# Autodesk Inventor assembly: Assembly1
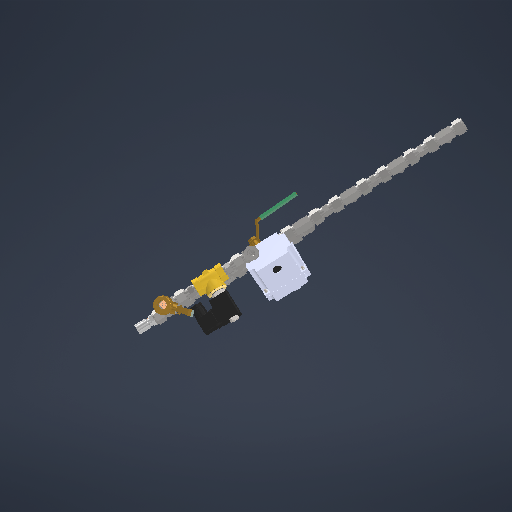
[picture p0: Inventor's stored thumbnail of the model, 512x512]
Saved by Autodesk Inventor 2026.2 (Build 302298000, 298)
## iProperties
Created: 2026-01-25
Part Number: Assembly1
Document SubType Name: Assembly
Designer: szwed
Author: szwed
## Documents named in this file (9)
- C:\Users\szwed\Desktop\R7\Assembly1.iam
- C:\Users\szwed\Documents\Inventor\Content Center Files\R2026\en-US\ISO 49 N8\ISO 49 Hexagon Nipple N8 3_8.ipt
- C:\Users\szwed\Documents\Inventor\Content Center Files\R2026\en-US\Parker A(16)\Parker A-Lok - Fractional Tube 1_2 (4).ipt
- C:\Users\szwed\Documents\Inventor\Content Center Files\R2026\en-US\Parker A(01)\Parker A-Lok - Metric to Inch Tube 12 x 1_2.ipt
- C:\Users\szwed\Documents\Inventor\Content Center Files\R2026\en-US\Parker A-Lok - 90deg Elbow - Fractional Tube\1_2(37).ipt
- C:\Users\szwed\Desktop\gs_solidworks-master\R7_GS_1110_SERVOVALVE\R7_GS_1110_SERVOVALVE\R7_GS_1110_SERVOVALVE\R7_GS_1110_SERVOVALVE.ipt
- C:\Users\szwed\Documents\Inventor\Content Center Files\R2026\en-US\Parker XV500P\Parker Female-Female Pipe Ends XV500P XV500P-8.ipt
- C:\Users\szwed\Documents\Inventor\Content Center Files\R2026\en-US\Parker MTT 2\Parker Male Taper Thread 1_4 x 3_8.ipt
- C:\Users\szwed\Downloads\MV04_DN8_3-8 Zoll\MV04_DN8_3-8 Zoll\MV04_DN8_3-8 Zoll.ipt
## Components (38 placed, 8 different names)
1. ISO 49 Hexagon Nipple N8 3/8:1 — Insert:7, Insert:8
2. Parker A-Lok - Fractional Tube 1/2:1 — Insert:2, Flush:1, Insert:3, Flush:2
3. ISO 49 Hexagon Nipple N8 3/8:5 — Insert:5, Insert:6
4. Parker A-Lok - Fractional Tube 1/2:2 — Insert:10, Flush:4, Insert:12, Insert:22, Flush:5, Flush:6
5. ISO 49 Hexagon Nipple N8 3/8:6 — Insert:15, Insert:17
6. Parker A-Lok - Fractional Tube 1/2:3 — Insert:4, Insert:5, Flush:2, Flush:3
7. ISO 49 Hexagon Nipple N8 3/8:7 — Insert:1, Insert:2
8. Parker A-Lok - Fractional Tube 1/2:4 — Insert:1, Flush:1
9. Parker A-Lok - Metric to Inch Tube 12 x 1/2:1 — Insert:13, Insert:15
10. ISO 49 Hexagon Nipple N8 3/8:8 — Insert:31, Insert:32
11. ISO 49 Hexagon Nipple N8 3/8:9 — Insert:11, Insert:13
12. Parker A-Lok - 90° Elbow - Fractional Tube 1/2:1 — Insert:17, Insert:18
13. R7_GS_1110_SERVOVALVE:1 — Insert:8, Insert:9
14. ISO 49 Hexagon Nipple N8 3/8:10 — Insert:3, Insert:4
15. Parker A-Lok - Metric to Inch Tube 12 x 1/2:2 — Insert:30, Insert:33
16. ISO 49 Hexagon Nipple N8 3/8:12 — Insert:29, Insert:30
17. ISO 49 Hexagon Nipple N8 3/8:13 — Insert:20, Insert:21
18. Parker A-Lok - 90° Elbow - Fractional Tube 1/2:2 — Insert:21, Flush:8, Insert:37, Insert:38
19. Parker A-Lok - Fractional Tube 1/2:5 — Insert:6, Flush:3, Insert:7, Flush:4, Insert:11, Flush:5
20. Parker Female-Female Pipe Ends XV500P XV500P-8:1 — Insert:19, Insert:20
21. ISO 49 Hexagon Nipple N8 3/8:14 — Insert:22, Insert:23
22. ISO 49 Hexagon Nipple N8 3/8:15 — Insert:12, Insert:14
23. ISO 49 Hexagon Nipple N8 3/8:16 — Insert:33, Insert:34
24. Parker A-Lok - Fractional Tube 1/2:6 — Insert:28, Flush:7, Insert:29, Insert:31, Flush:9
25. ISO 49 Hexagon Nipple N8 3/8:17 — Insert:35, Insert:36
26. Parker A-Lok - Metric to Inch Tube 12 x 1/2:3 — Insert:26, Insert:27
27. ISO 49 Hexagon Nipple N8 3/8:18 — Insert:38
28. Parker A-Lok - Fractional Tube 1/2:7 — Insert:23, Flush:6, Insert:24, Insert:25, Flush:7
29. ISO 49 Hexagon Nipple N8 3/8:19 — Insert:25, Insert:26
30. Parker Female-Female Pipe Ends XV500P XV500P-8:2 — Insert:34
31. Parker Male Taper Thread 1/4 x 3/8:1 — Insert:24
32. MV04_DN8_3-8 Zoll:1 — Insert:32, Insert:35
33. ISO 49 Hexagon Nipple N8 3/8:20 — Insert:27, Insert:28
34. ISO 49 Hexagon Nipple N8 3/8:21 — Insert:16, Insert:37
35. Parker A-Lok - 90° Elbow - Fractional Tube 1/2:3 — Insert:36, Flush:9
36. Parker A-Lok - Metric to Inch Tube 12 x 1/2:4 — Insert:14, Insert:16, Flush:8
37. ISO 49 Hexagon Nipple N8 3/8:22 — Insert:9, Insert:10
38. ISO 49 Hexagon Nipple N8 3/8:23 — Insert:18, Insert:19
## Relationships (47: Insert 38, Flush 9)
- Insert:1: ISO 49 Hexagon Nipple N8 3/8:7 ↔ Parker A-Lok - Fractional Tube 1/2:4
- Insert:2: Parker A-Lok - Fractional Tube 1/2:1 ↔ ISO 49 Hexagon Nipple N8 3/8:7
- Flush:1: Parker A-Lok - Fractional Tube 1/2:1 ↔ Parker A-Lok - Fractional Tube 1/2:4
- Insert:3: Parker A-Lok - Fractional Tube 1/2:1 ↔ ISO 49 Hexagon Nipple N8 3/8:10
- Insert:4: Parker A-Lok - Fractional Tube 1/2:3 ↔ ISO 49 Hexagon Nipple N8 3/8:10
- Insert:5: ISO 49 Hexagon Nipple N8 3/8:5 ↔ Parker A-Lok - Fractional Tube 1/2:3
- Insert:6: ISO 49 Hexagon Nipple N8 3/8:5 ↔ Parker A-Lok - Fractional Tube 1/2:5
- Flush:2: Parker A-Lok - Fractional Tube 1/2:1 ↔ Parker A-Lok - Fractional Tube 1/2:3
- Flush:3: Parker A-Lok - Fractional Tube 1/2:3 ↔ Parker A-Lok - Fractional Tube 1/2:5
- Insert:7: ISO 49 Hexagon Nipple N8 3/8:1 ↔ Parker A-Lok - Fractional Tube 1/2:5
- Insert:8: ISO 49 Hexagon Nipple N8 3/8:1 ↔ R7_GS_1110_SERVOVALVE:1
- Insert:9: R7_GS_1110_SERVOVALVE:1 ↔ ISO 49 Hexagon Nipple N8 3/8:22
- Insert:10: Parker A-Lok - Fractional Tube 1/2:2 ↔ ISO 49 Hexagon Nipple N8 3/8:22
- Flush:4: Parker A-Lok - Fractional Tube 1/2:2 ↔ Parker A-Lok - Fractional Tube 1/2:5
- Insert:11: ISO 49 Hexagon Nipple N8 3/8:9 ↔ Parker A-Lok - Fractional Tube 1/2:5
- Insert:12: Parker A-Lok - Fractional Tube 1/2:2 ↔ ISO 49 Hexagon Nipple N8 3/8:15
- Insert:13: Parker A-Lok - Metric to Inch Tube 12 x 1/2:1 ↔ ISO 49 Hexagon Nipple N8 3/8:9
- Insert:14: ISO 49 Hexagon Nipple N8 3/8:15 ↔ Parker A-Lok - Metric to Inch Tube 12 x 1/2:4
- Insert:15: ISO 49 Hexagon Nipple N8 3/8:6 ↔ Parker A-Lok - Metric to Inch Tube 12 x 1/2:1
- Insert:16: ISO 49 Hexagon Nipple N8 3/8:21 ↔ Parker A-Lok - Metric to Inch Tube 12 x 1/2:4
- Insert:17: ISO 49 Hexagon Nipple N8 3/8:6 ↔ Parker A-Lok - 90° Elbow - Fractional Tube 1/2:1
- Insert:18: Parker A-Lok - 90° Elbow - Fractional Tube 1/2:1 ↔ ISO 49 Hexagon Nipple N8 3/8:23
- Insert:19: Parker Female-Female Pipe Ends XV500P XV500P-8:1 ↔ ISO 49 Hexagon Nipple N8 3/8:23
- Insert:20: ISO 49 Hexagon Nipple N8 3/8:13 ↔ Parker Female-Female Pipe Ends XV500P XV500P-8:1
- Insert:21 (-10 mm): ISO 49 Hexagon Nipple N8 3/8:13 ↔ Parker A-Lok - 90° Elbow - Fractional Tube 1/2:2
- Insert:22: Parker A-Lok - Fractional Tube 1/2:2 ↔ ISO 49 Hexagon Nipple N8 3/8:14
- Flush:5: Parker A-Lok - Fractional Tube 1/2:2 ↔ Parker A-Lok - Fractional Tube 1/2:5
- Insert:23: ISO 49 Hexagon Nipple N8 3/8:14 ↔ Parker A-Lok - Fractional Tube 1/2:7
- Flush:6: Parker A-Lok - Fractional Tube 1/2:2 ↔ Parker A-Lok - Fractional Tube 1/2:7
- Insert:24: Parker A-Lok - Fractional Tube 1/2:7 ↔ Parker Male Taper Thread 1/4 x 3/8:1
- Insert:25: Parker A-Lok - Fractional Tube 1/2:7 ↔ ISO 49 Hexagon Nipple N8 3/8:19
- Insert:26: Parker A-Lok - Metric to Inch Tube 12 x 1/2:3 ↔ ISO 49 Hexagon Nipple N8 3/8:19
- Insert:27: Parker A-Lok - Metric to Inch Tube 12 x 1/2:3 ↔ ISO 49 Hexagon Nipple N8 3/8:20
- Insert:28: Parker A-Lok - Fractional Tube 1/2:6 ↔ ISO 49 Hexagon Nipple N8 3/8:20
- Flush:7: Parker A-Lok - Fractional Tube 1/2:6 ↔ Parker A-Lok - Fractional Tube 1/2:7
- Flush:8: Parker A-Lok - 90° Elbow - Fractional Tube 1/2:2 ↔ Parker A-Lok - Metric to Inch Tube 12 x 1/2:4
- Insert:29: ISO 49 Hexagon Nipple N8 3/8:12 ↔ Parker A-Lok - Fractional Tube 1/2:6
- Insert:30: Parker A-Lok - Metric to Inch Tube 12 x 1/2:2 ↔ ISO 49 Hexagon Nipple N8 3/8:12
- Insert:31: ISO 49 Hexagon Nipple N8 3/8:8 ↔ Parker A-Lok - Fractional Tube 1/2:6
- Insert:32: ISO 49 Hexagon Nipple N8 3/8:8 ↔ MV04_DN8_3-8 Zoll:1
- Insert:33: Parker A-Lok - Metric to Inch Tube 12 x 1/2:2 ↔ ISO 49 Hexagon Nipple N8 3/8:16
- Insert:34: ISO 49 Hexagon Nipple N8 3/8:16 ↔ Parker Female-Female Pipe Ends XV500P XV500P-8:2
- Insert:35: ISO 49 Hexagon Nipple N8 3/8:17 ↔ MV04_DN8_3-8 Zoll:1
- Insert:36: ISO 49 Hexagon Nipple N8 3/8:17 ↔ Parker A-Lok - 90° Elbow - Fractional Tube 1/2:3
- Flush:9: Parker A-Lok - Fractional Tube 1/2:6 ↔ Parker A-Lok - 90° Elbow - Fractional Tube 1/2:3
- Insert:37: Parker A-Lok - 90° Elbow - Fractional Tube 1/2:2 ↔ ISO 49 Hexagon Nipple N8 3/8:21
- Insert:38: Parker A-Lok - 90° Elbow - Fractional Tube 1/2:2 ↔ ISO 49 Hexagon Nipple N8 3/8:18
